# Autodesk Inventor assembly: Montagem2
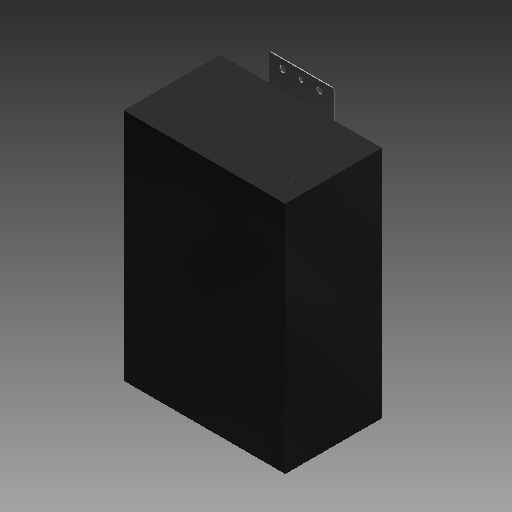
[picture p0: Inventor's stored thumbnail of the model, 512x512]
Saved by Autodesk Inventor 2019.4 (Build 234330000, 330)
## iProperties
Created: 2020-12-12
Part Number: Montagem2
Material: Genérico
Document SubType Name: Assembly
Designer: Lattes
Author: Lattes
## Documents named in this file (24)
- D:\Lattes\Documents\GitHub-HD\estacao-meteorologica-it\Estuturas\caixa\caixa de instrumentação e controle.iam
- D:\Lattes\Documents\GitHub-HD\estacao-meteorologica-it\Estuturas\caixa\base da caixa.ipt
- D:\Lattes\Documents\GitHub-HD\estacao-meteorologica-it\Estuturas\caixa\fixador bateria v2.5 - R.ipt
- D:\Lattes\Documents\GitHub-HD\estacao-meteorologica-it\Estuturas\caixa\bateria 12mva-7.ipt
- D:\Lattes\Documents\GitHub-HD\estacao-meteorologica-it\Estuturas\caixa\fixador bateria v2.5 - L.ipt
- D:\Lattes\Documents\GitHub-HD\estacao-meteorologica-it\Estuturas\caixa\controlador solar v1.ipt
- D:\Lattes\Documents\GitHub-HD\estacao-meteorologica-it\Estuturas\caixa\Encaixe suporte controlador.ipt
- D:\Lattes\Documents\GitHub-HD\estacao-meteorologica-it\Estuturas\caixa\respirador_v1.ipt
- D:\Lattes\Documents\GitHub-HD\estacao-meteorologica-it\Estuturas\caixa\borracha isolamento respirador.ipt
- D:\Lattes\Documents\GitHub-HD\estacao-meteorologica-it\Estuturas\caixa\Parafuso m3 15mm.ipt
- D:\Lattes\Documents\GitHub-HD\estacao-meteorologica-it\Estuturas\caixa\porca m3.ipt
- D:\Lattes\Documents\GitHub-HD\estacao-meteorologica-it\Estuturas\caixa\borracha isolamento prensa cabo.ipt
- D:\Lattes\Documents\GitHub-HD\estacao-meteorologica-it\Estuturas\caixa\Prensa cabo fixador.ipt
- D:\Lattes\Documents\GitHub-HD\estacao-meteorologica-it\Estuturas\caixa\Chapa fixação caixa.ipt
- D:\Lattes\Documents\GitHub-HD\estacao-meteorologica-it\Estuturas\caixa\ruela m6 borracha.ipt
- D:\Lattes\Documents\GitHub-HD\estacao-meteorologica-it\Estuturas\caixa\ruela m6.ipt
- D:\Lattes\Documents\GitHub-HD\estacao-meteorologica-it\Estuturas\caixa\tampa caixa.ipt
- D:\Lattes\Documents\GitHub-HD\estacao-meteorologica-it\Estuturas\caixa\espaçador 15mm m3.ipt
- D:\Lattes\Documents\GitHub-HD\estacao-meteorologica-it\Estuturas\caixa\Fixador caixa-tubo.ipt
- D:\Lattes\Documents\GitHub-HD\estacao-meteorologica-it\Estuturas\caixa\parafuso 1 quarto 16mm.ipt
- D:\Lattes\Documents\GitHub-HD\estacao-meteorologica-it\Estuturas\caixa\porca 1 quarto.ipt
- D:\Lattes\Documents\GitHub-HD\estacao-meteorologica-it\Estuturas\caixa\anel de borracha para m6.ipt
- D:\Lattes\Documents\GitHub-HD\estacao-meteorologica-it\Estuturas\caixa\ruela m3.ipt
- D:\Lattes\Documents\GitHub-HD\estacao-meteorologica-it\Estuturas\caixa\Parafuso m3 6mm.ipt
## Components (53 placed, 23 different names)
1. base da caixa:1 — Inserir:1, Coincidência:3, Coincidência:4, Inserir:2, Inserir:4, Inserir:6, Inserir:7, Inserir:8, Inserir:12, Inserir:13, Inserir:20, Inserir:21, Inserir:22, Inserir:23, Inserir:40, Inserir:41, Inserir:70, Inserir:71, Coincidência:7, Coincidência:8, Inserir:81, Inserir:82, Inserir:83, Inserir:84, Inserir:89, Inserir:90
2. fixador bateria v2.5 - R:1 — Inserir:1, Coincidência:1, Coincidência:2, Tangente:1, Coincidência:5, Coincidência:6, Rígida:1, Inserir:93
3. bateria 12mva-7:1 — Coincidência:1, Coincidência:2, Coincidência:3, Coincidência:4
4. fixador bateria v2.5 - L:1 — Inserir:2, Inserir:3, Rígida:2, Inserir:94
5. controlador solar v1:1 — Tangente:1, Coincidência:5, Coincidência:6
6. Encaixe suporte controlador:1 — Inserir:3
7. respirador_v1:1 — Inserir:4, Inserir:5, Inserir:9, Inserir:10, Inserir:11
8. borracha isolamento respirador:1 — Inserir:5
9. Parafuso m3 15mm:1 — Inserir:6
10. Parafuso m3 15mm:2 — Inserir:8
11. Parafuso m3 15mm:3 — Inserir:7
12. porca m3:1 — Inserir:9
13. porca m3:2 — Inserir:11
14. porca m3:3 — Inserir:10
15. borracha isolamento prensa cabo:1 — Inserir:12, Inserir:14
16. borracha isolamento prensa cabo:2 — Inserir:13, Inserir:15
17. Prensa cabo fixador:1 — Inserir:14, Inserir:18, Inserir:19
18. Prensa cabo fixador:2 — Inserir:15, Inserir:16, Inserir:17
19. Parafuso m3 15mm:4 — Inserir:18
20. porca m3:4 — Inserir:22
21. Parafuso m3 15mm:5 — Inserir:19
22. porca m3:5 — Inserir:23
23. Parafuso m3 15mm:6 — Inserir:17
24. porca m3:6 — Inserir:21
25. Parafuso m3 15mm:7 — Inserir:16
26. porca m3:7 — Inserir:20
27. ruela m6 borracha:3 — Inserir:69, Inserir:85
28. ruela m6 borracha:4 — Inserir:68, Inserir:86
29. ruela m6 borracha:5 — Inserir:43, Inserir:87
30. ruela m6 borracha:8 — Inserir:42, Inserir:88
31. ruela m6:1 — Inserir:41, Inserir:43
32. ruela m6:2 — Inserir:40, Inserir:42
33. Chapa fixação caixa:1 — Inserir:68, Inserir:69, Inserir:70, Inserir:71
34. tampa caixa:2 — Coincidência:7, Coincidência:8
35. espaçador 15mm m3:1 — Inserir:81, Inserir:97
36. espaçador 15mm m3:2 — Inserir:82, Inserir:95
37. espaçador 15mm m3:3 — Inserir:83, Inserir:96
38. Fixador caixa-tubo:1 — Inserir:84
39. parafuso 1 quarto 16mm:1 — Inserir:85
40. parafuso 1 quarto 16mm:2 — Inserir:86
41. porca 1 quarto:1 — Inserir:87
42. porca 1 quarto:2 — Inserir:88
43. anel de borracha para m6:1 — Rígida:1
44. anel de borracha para m6:2 — Rígida:2
45. ruela m3:1 — Inserir:89, Inserir:91
46. ruela m3:2 — Inserir:90, Inserir:92
47. Parafuso m3 6mm:1 — Inserir:96
48. Parafuso m3 6mm:2 — Inserir:94
49. Parafuso m3 6mm:3 — Inserir:97
50. Parafuso m3 6mm:4 — Inserir:91
51. Parafuso m3 6mm:5 — Inserir:92
52. Parafuso m3 6mm:6 — Inserir:93
53. Parafuso m3 6mm:7 — Inserir:95
## Relationships (59: Insert 48, Mate 8, WeldJoint 2, Tangent 1)
- Inserir:1 (-5 mm): base da caixa:1 ↔ fixador bateria v2.5 - R:1
- Coincidência:1 [Mate] (1 mm): fixador bateria v2.5 - R:1 ↔ bateria 12mva-7:1
- Coincidência:2 [Mate]: fixador bateria v2.5 - R:1 ↔ bateria 12mva-7:1
- Coincidência:3 [Mate] (1 mm): base da caixa:1 ↔ bateria 12mva-7:1
- Coincidência:4 [Mate] (0.5 mm): base da caixa:1 ↔ bateria 12mva-7:1
- Inserir:2: base da caixa:1 ↔ fixador bateria v2.5 - L:1
- Tangente:1: fixador bateria v2.5 - R:1 ↔ controlador solar v1:1
- Coincidência:5 [Mate]: fixador bateria v2.5 - R:1 ↔ controlador solar v1:1
- Inserir:3 (-3 mm): fixador bateria v2.5 - L:1 ↔ Encaixe suporte controlador:1
- Coincidência:6 [Mate]: fixador bateria v2.5 - R:1 ↔ controlador solar v1:1
- Inserir:4 (1 mm): base da caixa:1 ↔ respirador_v1:1
- Inserir:5: respirador_v1:1 ↔ borracha isolamento respirador:1
- Inserir:6: base da caixa:1 ↔ Parafuso m3 15mm:1
- Inserir:7: base da caixa:1 ↔ Parafuso m3 15mm:3
- Inserir:8: base da caixa:1 ↔ Parafuso m3 15mm:2
- Inserir:9: respirador_v1:1 ↔ porca m3:1
- Inserir:10: respirador_v1:1 ↔ porca m3:3
- Inserir:11: respirador_v1:1 ↔ porca m3:2
- Inserir:12: base da caixa:1 ↔ borracha isolamento prensa cabo:1
- Inserir:13: base da caixa:1 ↔ borracha isolamento prensa cabo:2
- Inserir:14: borracha isolamento prensa cabo:1 ↔ Prensa cabo fixador:1
- Inserir:15: borracha isolamento prensa cabo:2 ↔ Prensa cabo fixador:2
- Inserir:16: Prensa cabo fixador:2 ↔ Parafuso m3 15mm:7
- Inserir:17: Prensa cabo fixador:2 ↔ Parafuso m3 15mm:6
- Inserir:18: Prensa cabo fixador:1 ↔ Parafuso m3 15mm:4
- Inserir:19: Prensa cabo fixador:1 ↔ Parafuso m3 15mm:5
- Inserir:20: base da caixa:1 ↔ porca m3:7
- Inserir:21: base da caixa:1 ↔ porca m3:6
- Inserir:22: base da caixa:1 ↔ porca m3:4
- Inserir:23: base da caixa:1 ↔ porca m3:5
- Inserir:40: base da caixa:1 ↔ ruela m6:2
- Inserir:41: base da caixa:1 ↔ ruela m6:1
- Inserir:42: ruela m6 borracha:8 ↔ ruela m6:2
- Inserir:43: ruela m6 borracha:5 ↔ ruela m6:1
- Inserir:68: ruela m6 borracha:4 ↔ Chapa fixação caixa:1
- Inserir:69: ruela m6 borracha:3 ↔ Chapa fixação caixa:1
- Inserir:70: base da caixa:1 ↔ Chapa fixação caixa:1
- Inserir:71: base da caixa:1 ↔ Chapa fixação caixa:1
- Coincidência:7 [Mate]: base da caixa:1 ↔ tampa caixa:2
- Coincidência:8 [Mate]: base da caixa:1 ↔ tampa caixa:2
- Inserir:81: base da caixa:1 ↔ espaçador 15mm m3:1
- Inserir:82: base da caixa:1 ↔ espaçador 15mm m3:2
- Inserir:83: base da caixa:1 ↔ espaçador 15mm m3:3
- Inserir:84: base da caixa:1 ↔ Fixador caixa-tubo:1
- Inserir:85: ruela m6 borracha:3 ↔ parafuso 1 quarto 16mm:1
- Inserir:86: ruela m6 borracha:4 ↔ parafuso 1 quarto 16mm:2
- Inserir:87: ruela m6 borracha:5 ↔ porca 1 quarto:1
- Inserir:88: ruela m6 borracha:8 ↔ porca 1 quarto:2
- Rígida:1 [WeldJoint] (0.74 mm): fixador bateria v2.5 - R:1 ↔ anel de borracha para m6:1
- Rígida:2 [WeldJoint] (-0.74 mm): fixador bateria v2.5 - L:1 ↔ anel de borracha para m6:2
- Inserir:89: base da caixa:1 ↔ ruela m3:1
- Inserir:90: base da caixa:1 ↔ ruela m3:2
- Inserir:91: ruela m3:1 ↔ Parafuso m3 6mm:4
- Inserir:92: ruela m3:2 ↔ Parafuso m3 6mm:5
- Inserir:93: fixador bateria v2.5 - R:1 ↔ Parafuso m3 6mm:6
- Inserir:94: fixador bateria v2.5 - L:1 ↔ Parafuso m3 6mm:2
- Inserir:95: espaçador 15mm m3:2 ↔ Parafuso m3 6mm:7
- Inserir:96: espaçador 15mm m3:3 ↔ Parafuso m3 6mm:1
- Inserir:97: espaçador 15mm m3:1 ↔ Parafuso m3 6mm:3
